# Autodesk Inventor assembly: ASY MSC 002 отстойник осветлитель
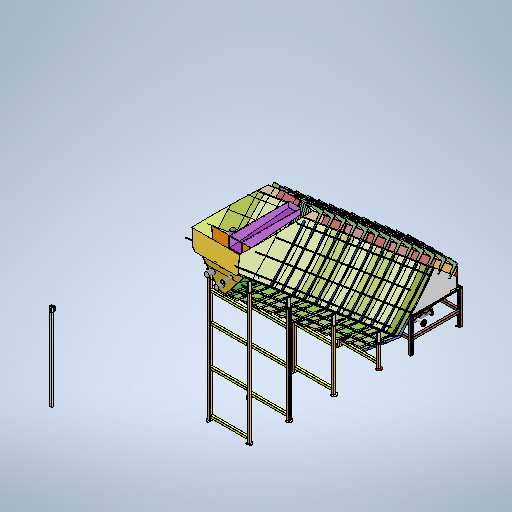
[picture p0: Inventor's stored thumbnail of the model, 512x512]
Saved by Autodesk Inventor 2025 (Build 290162010, 162A)
## iProperties
Created: 2024-09-05
Part Number: ASY MSC 002 отстойник осветлитель
Document SubType Name: Assembly
Designer: admin
Author: admin
## Documents named in this file (42)
- C:\Users\pokla\Documents\Inventor\Manturovo2\ASY MSC 002 отстойник осветлитель.iam
- C:\Users\pokla\Documents\Inventor\Manturovo2\ASY MSC 900.1 base frame.iam
- C:\Users\pokla\Documents\Inventor\Manturovo2\ASY MSC 100 cone.iam
- C:\Users\pokla\Documents\Inventor\Manturovo2\MSC 401 sheet lowerback.ipt
- C:\Users\pokla\Documents\Inventor\Manturovo2\MSC 313 sheet left board hip.ipt
- C:\Users\pokla\Documents\Inventor\Manturovo2\MSC 312 sheet right board hip.ipt
- C:\Users\pokla\Documents\Inventor\Manturovo2\MSC 706 ridge 1.ipt
- C:\Users\pokla\Documents\Inventor\Manturovo2\MSC 701 face 1.ipt
- C:\Users\pokla\Documents\Inventor\Manturovo2\MSC 705 ridge 3.ipt
- C:\Users\pokla\Documents\Inventor\Manturovo2\MSC 713 tube.ipt
- C:\Users\pokla\Documents\Inventor\Manturovo2\ISO 5251 Bends 3D without straight ends(90 deg) DN150 11 11.ipt
- C:\Users\pokla\Documents\Inventor\Manturovo2\MSC 712 tube.ipt
- C:\Users\pokla\Documents\Inventor\Manturovo2\MSC 711 tube.ipt
- C:\Users\pokla\Documents\Inventor\Manturovo2\MSC 408 stringer lowerback.ipt
- C:\Users\pokla\Documents\Inventor\Manturovo2\MSC 707 ridge 2.ipt
- C:\Users\pokla\Documents\Inventor\Manturovo2\MSC 703 face 2.ipt
- C:\Users\pokla\Documents\Inventor\Manturovo2\MSC 702 face 3.ipt
- C:\Users\pokla\Documents\Inventor\Manturovo2\MSC 704 face 4.ipt
- C:\Users\pokla\Documents\Inventor\Manturovo2\MSC 708 ridge 4.ipt
- C:\Users\pokla\Documents\Inventor\Manturovo2\MSC 709 ridge 5.ipt
- C:\Users\pokla\Documents\Inventor\Manturovo2\ASY MSC 900.3 base frame.iam
- C:\Users\pokla\Documents\Inventor\Manturovo2\Pillars\ASY MSC 900.5 base frame.iam
- C:\Users\pokla\Documents\Inventor\Manturovo2\Pillars\ASY MSC 900.4  base frame.iam
- C:\Users\pokla\Documents\Inventor\Manturovo2\Pillars\ASY MSC 900.6 base frame.iam
- C:\Users\pokla\Documents\Inventor\Manturovo2\ASY MSC 200 BACK.iam
- C:\Users\pokla\Documents\Inventor\Manturovo2\ASY MSC 300.2 LEFT BOARD.iam
- C:\Users\pokla\Documents\Inventor\Manturovo2\ASY MSC 300.1 RIGHT BOARD.iam
- C:\Users\pokla\Documents\Inventor\Manturovo2\ASY MSC 500 BELLY.iam
- C:\Users\pokla\Documents\Inventor\Manturovo2\MSC 316 stringer board #.ipt
- C:\Users\pokla\Documents\Inventor\Manturovo2\MSC 317 stringer board ##.ipt
- C:\Users\pokla\Documents\Inventor\Manturovo2\MSC 315 rib hip.ipt
- C:\Users\pokla\Documents\Inventor\Manturovo2\MSC 314 rib hip.ipt
- C:\Users\pokla\Documents\Inventor\Manturovo2\ASY MSC 900.2 support.iam
- C:\Users\pokla\Documents\Inventor\Manturovo2\ASY MSC 600 cone exit back.iam
- C:\Users\pokla\Documents\Inventor\Manturovo2\MSC 710 flange.ipt
- C:\Users\pokla\Documents\Inventor\Manturovo2\ASY MSC 800 gills.iam
- C:\Users\pokla\Documents\Inventor\Manturovo2\MSC 407 sheet lowerback_FIX.ipt
- C:\Users\pokla\Documents\Inventor\Manturovo2\ASY MSC 400 Accsess hatch.iam
- C:\Users\pokla\Documents\Inventor\Manturovo2\MSC DIM 000 settler-clarifier.ipt
- C:\Users\pokla\Documents\Inventor\Manturovo2\MSC DIM 001 frame.ipt
- C:\Users\pokla\Documents\Inventor\Manturovo2\MSC 908 transverse pillar plate.ipt
- C:\Users\pokla\Documents\Inventor\Manturovo2\MSC 907 transverse pipe.ipt
## Components (54 placed, 41 different names)
1. MSC DIM 000 settler-clarifier.ipt:1
2. MSC DIM 001 frame.ipt:1
3. ASY MSC 900.1 base frame.iam:1 [sub-assembly] — Flush:4, Mate:18, Flush:5, Mate:19, Mate:44, Mate:47
4. ASY MSC 100 cone.iam:1 [sub-assembly] — Mate:19, Flush:6, Mate:27, Mate:29
5. MSC 401 sheet lowerback.ipt:1 — Mate:29, Mate:30, Mate:31
6. MSC 313 sheet left board hip.ipt:1 — Mate:27
7. MSC 312 sheet right board hip.ipt:1
8. MSC 706 ridge 1.ipt:1
9. MSC 701 face 1.ipt:1 — Flush:9, Mate:35
10. MSC 705 ridge 3.ipt:1 — Rigid:12, Rigid:14
11. MSC 713 tube.ipt:1
12. ISO 5251 Bends 3D without straight ends(90 deg) DN150 11 11.ipt:1
13. MSC 712 tube.ipt:1
14. MSC 711 tube.ipt:1
15. MSC 408 stringer lowerback.ipt:1
16. MSC 707 ridge 2.ipt:1 — Rigid:12, Rigid:13
17. MSC 713 tube.ipt:2
18. MSC 703 face 2.ipt:1 — Mate:37, Flush:12, Flush:13
19. MSC 702 face 3.ipt:1 — Mate:34, Mate:35, Mate:36
20. MSC 704 face 4.ipt:1
21. MSC 408 stringer lowerback.ipt:2
22. MSC 708 ridge 4.ipt:1 — Rigid:14
23. MSC 709 ridge 5.ipt:1 — Rigid:13
24. ASY MSC 900.3 base frame.iam:1 [sub-assembly] — Mate:23, Mate:24, Cylindrical:4, Mate:44, Mate:45
25. ASY MSC 900.5 base frame.iam:1 [sub-assembly] — Flush:10, Flush:11, Cylindrical:7, Cylindrical:8, Mate:46
26. ASY MSC 900.4  base frame.iam:1 [sub-assembly] — Mate:32, Mate:33, Mate:45, Mate:46
27. ASY MSC 900.6 base frame.iam:1 [sub-assembly] — Mate:38, Mate:39, Cylindrical:5, Cylindrical:6, Mate:47
28. ASY MSC 200 BACK.iam:1 [sub-assembly] — Flush:8, Mate:31
29. ASY MSC 300.2 LEFT BOARD.iam:1 [sub-assembly] — Rigid:11, Mate:34, Flush:12
30. ASY MSC 300.1 RIGHT BOARD.iam:1 [sub-assembly] — Rigid:10, Mate:37
31. ASY MSC 500 BELLY.iam:1 [sub-assembly] — Flush:7, Mate:22, Mate:25, Rigid:10, Rigid:11, Mate:40, Mate:41, Mate:42, Mate:43
32. MSC 316 stringer board #.ipt:1
33. MSC 317 stringer board ##.ipt:1
34. MSC 315 rib hip.ipt:1
35. MSC 314 rib hip.ipt:1
36. MSC 316 stringer board #.ipt:2
37. MSC 317 stringer board ##.ipt:2
38. MSC 315 rib hip.ipt:2
39. MSC 314 rib hip.ipt:2
40. ASY MSC 900.2 support.iam:1 [sub-assembly] — Cylindrical:8, Mate:40
41. ASY MSC 900.2 support.iam:2 [sub-assembly]
42. ASY MSC 900.2 support.iam:3 [sub-assembly] — Cylindrical:4, Mate:25
43. ASY MSC 900.2 support.iam:4 [sub-assembly] — Cylindrical:6, Mate:42
44. ASY MSC 900.2 support.iam:5 [sub-assembly]
45. ASY MSC 600 cone exit back.iam:1 [sub-assembly]
46. MSC 710 flange.ipt:1
47. ASY MSC 800 gills.iam:1 [sub-assembly] — Mate:22
48. MSC 407 sheet lowerback_FIX.ipt:1
49. ASY MSC 900.2 support.iam:6 [sub-assembly] — Cylindrical:7, Mate:41
50. ASY MSC 900.2 support.iam:7 [sub-assembly]
51. ASY MSC 400 Accsess hatch.iam:1 [sub-assembly]
52. ASY MSC 900.2 support.iam:8 [sub-assembly] — Cylindrical:5, Mate:43
53. MSC 907 transverse pipe.ipt:1
54. MSC 908 transverse pillar plate.ipt:1
## Relationships (72: Mate 37, WeldJoint 13, Flush 13, CylindricalJoint 8, RevoluteJoint 1)
- [Mate]: ASY MSC 100 cone.iam:1 ↔ MSC 401 sheet lowerback.ipt:1
- [WeldJoint]: MSC 713 tube.ipt:1 ↔ ISO 5251 Bends 3D without straight ends(90 deg) DN150 11 11.ipt:1
- [Mate]: ASY MSC 100 cone.iam:1 ↔ MSC 408 stringer lowerback.ipt:1
- [RevoluteJoint]: ISO 5251 Bends 3D without straight ends(90 deg) DN150 11 11.ipt:1 ↔ MSC 713 tube.ipt:2
- [WeldJoint]: MSC 701 face 1.ipt:1 ↔ MSC 712 tube.ipt:1
- [WeldJoint]: MSC 701 face 1.ipt:1 ↔ MSC 711 tube.ipt:1
- [WeldJoint] (-200 mm): MSC 701 face 1.ipt:1 ↔ MSC 713 tube.ipt:1
- [Mate]: ASY MSC 100 cone.iam:1 ↔ MSC 408 stringer lowerback.ipt:2
- [Mate]: ASY MSC 500 BELLY.iam:1 ↔ ASY MSC 600 cone exit back.iam:1
- [Flush]: ASY MSC 900.1 base frame.iam:1 ↔ ASY MSC 100 cone.iam:1
- [WeldJoint]: ASY MSC 100 cone.iam:1 ↔ ASY MSC 600 cone exit back.iam:1
- Rigid:12 [WeldJoint]: MSC 705 ridge 3.ipt:1 ↔ MSC 707 ridge 2.ipt:1
- [WeldJoint]: MSC 706 ridge 1.ipt:1 ↔ MSC 705 ridge 3.ipt:1
- [Flush]: ASY MSC 500 BELLY.iam:1 ↔ ASY MSC 600 cone exit back.iam:1
- [WeldJoint]: MSC 711 tube.ipt:1 ↔ MSC 710 flange.ipt:1
- [Mate]: ASY MSC 500 BELLY.iam:1 ↔ ASY MSC 800 gills.iam:1
- [Mate]: MSC 701 face 1.ipt:1 ↔ ASY MSC 500 BELLY.iam:1
- [Mate] (-5 mm): MSC 701 face 1.ipt:1 ↔ ASY MSC 500 BELLY.iam:1
- [Mate]: ASY MSC 500 BELLY.iam:1 ↔ ASY MSC 900.2 support.iam:2
- [Mate]: ASY MSC 500 BELLY.iam:1 ↔ ASY MSC 900.2 support.iam:5
- [Mate]: ASY MSC 500 BELLY.iam:1 ↔ ASY MSC 900.2 support.iam:7
- [CylindricalJoint]: ASY MSC 900.4  base frame.iam:1 ↔ ASY MSC 900.2 support.iam:5
- [CylindricalJoint]: ASY MSC 900.4  base frame.iam:1 ↔ ASY MSC 900.2 support.iam:2
- [Mate] (-2860 mm): ASY MSC 200 BACK.iam:1 ↔ ASY MSC 500 BELLY.iam:1
- [CylindricalJoint]: ASY MSC 900.3 base frame.iam:1 ↔ ASY MSC 900.2 support.iam:7
- [Flush]: ASY MSC 900.3 base frame.iam:1 ↔ ASY MSC 900.4  base frame.iam:1
- Flush:4: ASY MSC 900.1 base frame.iam:1
- Mate:18 (4 mm): ASY MSC 900.1 base frame.iam:1
- Flush:5: ASY MSC 900.1 base frame.iam:1
- Mate:19: ASY MSC 900.1 base frame.iam:1 ↔ ASY MSC 100 cone.iam:1
- Flush:6: ASY MSC 100 cone.iam:1
- Flush:7: ASY MSC 500 BELLY.iam:1
- Flush:8: ASY MSC 200 BACK.iam:1
- Mate:22: ASY MSC 500 BELLY.iam:1 ↔ ASY MSC 800 gills.iam:1
- Mate:23: ASY MSC 900.3 base frame.iam:1
- Mate:24: ASY MSC 900.3 base frame.iam:1
- Cylindrical:4: ASY MSC 900.3 base frame.iam:1 ↔ ASY MSC 900.2 support.iam:3
- Mate:25: ASY MSC 500 BELLY.iam:1 ↔ ASY MSC 900.2 support.iam:3
- Flush:9: MSC 701 face 1.ipt:1
- Mate:27: ASY MSC 100 cone.iam:1 ↔ MSC 313 sheet left board hip.ipt:1
- Mate:29: ASY MSC 100 cone.iam:1 ↔ MSC 401 sheet lowerback.ipt:1
- Mate:30: MSC 401 sheet lowerback.ipt:1
- Mate:31: MSC 401 sheet lowerback.ipt:1 ↔ ASY MSC 200 BACK.iam:1
- Rigid:10 [WeldJoint] (-25 mm): ASY MSC 300.1 RIGHT BOARD.iam:1 ↔ ASY MSC 500 BELLY.iam:1
- Rigid:11 [WeldJoint] (-25 mm): ASY MSC 300.2 LEFT BOARD.iam:1 ↔ ASY MSC 500 BELLY.iam:1
- Flush:10: ASY MSC 900.5 base frame.iam:1
- Flush:11: ASY MSC 900.5 base frame.iam:1
- Mate:32: ASY MSC 900.4  base frame.iam:1
- Mate:33: ASY MSC 900.4  base frame.iam:1
- Mate:34: MSC 702 face 3.ipt:1 ↔ ASY MSC 300.2 LEFT BOARD.iam:1
- Mate:35: MSC 701 face 1.ipt:1 ↔ MSC 702 face 3.ipt:1
- Rigid:13 [WeldJoint]: MSC 707 ridge 2.ipt:1 ↔ MSC 709 ridge 5.ipt:1
- Rigid:14 [WeldJoint]: MSC 705 ridge 3.ipt:1 ↔ MSC 708 ridge 4.ipt:1
- Mate:36: MSC 702 face 3.ipt:1
- Mate:37: MSC 703 face 2.ipt:1 ↔ ASY MSC 300.1 RIGHT BOARD.iam:1
- Mate:38: ASY MSC 900.6 base frame.iam:1
- Mate:39: ASY MSC 900.6 base frame.iam:1
- Cylindrical:5: ASY MSC 900.6 base frame.iam:1 ↔ ASY MSC 900.2 support.iam:8
- Cylindrical:6: ASY MSC 900.6 base frame.iam:1 ↔ ASY MSC 900.2 support.iam:4
- Cylindrical:7: ASY MSC 900.5 base frame.iam:1 ↔ ASY MSC 900.2 support.iam:6
- Cylindrical:8: ASY MSC 900.5 base frame.iam:1 ↔ ASY MSC 900.2 support.iam:1
- Mate:40 (3 mm): ASY MSC 500 BELLY.iam:1 ↔ ASY MSC 900.2 support.iam:1
- Mate:41 (3 mm): ASY MSC 500 BELLY.iam:1 ↔ ASY MSC 900.2 support.iam:6
- Mate:42: ASY MSC 500 BELLY.iam:1 ↔ ASY MSC 900.2 support.iam:4
- Mate:43 (3 mm): ASY MSC 500 BELLY.iam:1 ↔ ASY MSC 900.2 support.iam:8
- Flush:12: MSC 703 face 2.ipt:1 ↔ ASY MSC 300.2 LEFT BOARD.iam:1
- Flush:13: MSC 703 face 2.ipt:1
- Mate:44 (860 mm): ASY MSC 900.1 base frame.iam:1 ↔ ASY MSC 900.3 base frame.iam:1
- Mate:45 (1430 mm): ASY MSC 900.3 base frame.iam:1 ↔ ASY MSC 900.4  base frame.iam:1
- Mate:46 (1430 mm): ASY MSC 900.5 base frame.iam:1 ↔ ASY MSC 900.4  base frame.iam:1
- Mate:47 (5215 mm): ASY MSC 900.1 base frame.iam:1 ↔ ASY MSC 900.6 base frame.iam:1
- [WeldJoint]: MSC 907 transverse pipe.ipt:1 ↔ MSC 908 transverse pillar plate.ipt:1
